# Autodesk Inventor assembly: assembly
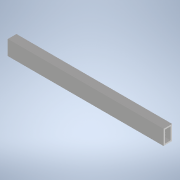
[picture p0: Inventor's stored thumbnail of the model, 180x180]
Saved by Autodesk Inventor 2022 (Build 260153000, 153)
## iProperties
Created: 2021-07-03
Part Number: assembly
Document SubType Name: Assembly
Designer: Ferdinand Hubbard
Author: Ferdinand Hubbard
## Documents named in this file (5)
- C:\Users\Ferdinand Hubbard\Desktop\solarplane\cad\easy bake oven\assembly.iam
- C:\Users\Ferdinand Hubbard\Desktop\solarplane\cad\easy bake oven\long.ipt
- C:\Users\Ferdinand Hubbard\Desktop\solarplane\cad\easy bake oven\short.ipt
- C:\Users\Ferdinand Hubbard\Desktop\solarplane\cad\30 mm tube.ipt
- C:\Users\Ferdinand Hubbard\Desktop\solarplane\cad\9mm tube.ipt
## Components (7 placed, 4 different names)
1. long:1 — Mate:2, Mate:3, Mate:5, Flush:1
2. long:2 — Mate:1, Mate:4
3. short:1 — Mate:1, Mate:2, Mate:3, Mate:4
4. short:2 — Mate:5, Flush:1
5. 30 mm tube:1
6. 30 mm tube:2
7. 9mm tube:1
## Relationships (6: Mate 5, Flush 1)
- Mate:1: long:2 ↔ short:1
- Mate:2: long:1 ↔ short:1
- Mate:3: long:1 ↔ short:1
- Mate:4: long:2 ↔ short:1
- Mate:5: long:1 ↔ short:2
- Flush:1: long:1 ↔ short:2
